# Autodesk Inventor assembly: 右後脚ユニット2
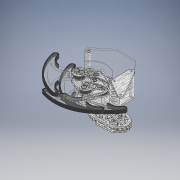
[picture p0: Inventor's stored thumbnail of the model, 180x180]
Saved by Autodesk Inventor 2020 (Build 240168000, 168)
## iProperties
Created: 2019-07-31
Part Number: 右後脚ユニット2
Document SubType Name: Assembly
Designer: 雪村
Mass: 201.521 g
Surface Area: 1076.65 cm^2
Volume: 97.0922 cm^3
Density: 2.07557 g/cm^3
Author: 雪村
## Documents named in this file (12)
- C:\Users\white\Documents\SRDC\SRDC\Inventor_2017\2018年機体\2020年4年機体\右後脚ユニット2.iam
- C:\Users\white\Documents\SRDC\SRDC\Inventor_2017\2018年機体\2020年4年機体\脚内フレーム1.ipt
- C:\Users\white\Documents\SRDC\SRDC\Inventor_2017\2018年機体\2020年4年機体\脚クランク1.iam
- C:\Users\white\Documents\SRDC\SRDC\Inventor_2017\2018年機体\パーツ\オイレスフランジ付き12142006.ipt
- C:\Users\white\Documents\SRDC\SRDC\Inventor_2017\2018年機体\2020年4年機体\脚最終段カム1.ipt
- C:\Users\white\Documents\SRDC\SRDC\Inventor_2017\2018年機体\2020年4年機体\歯車m2.z14.ipt
- C:\Users\white\Documents\SRDC\SRDC\Inventor_2017\2018年機体\パーツ\スペーサーm3,35.ipt
- C:\Users\white\Documents\SRDC\SRDC\Inventor_2017\2018年機体\2020年4年機体\ヘッケン＋揺動節1_MIR.iam
- C:\Users\white\Documents\SRDC\SRDC\Inventor_2017\2018年機体\2020年4年機体\脚外フレーム1.ipt
- C:\Users\white\Documents\SRDC\SRDC\Inventor_2017\2018年機体\2020年4年機体\後脚ギアトレイン1_MIR1.iam
- C:\Users\white\Documents\SRDC\SRDC\Inventor_2017\2018年機体\パーツ\オイレスフランジ付き14162202.5.ipt
- C:\Users\white\Documents\SRDC\SRDC\Inventor_2017\2018年機体\2020年4年機体\後脚ユニット締結パーツ2_MIR.ipt
## Components (16 placed, 11 different names)
1. 脚内フレーム1:1 — 挿入:9, 挿入:10, 挿入:11, 挿入:15, 挿入:18
2. 脚クランク1:1 [sub-assembly]
3. オイレスフランジ付き12142006:1 — 挿入:9
4. 脚最終段カム1:1
5. 歯車m2.z14:1
6. スペーサーm3,35:1 — 挿入:10, 挿入:13
7. スペーサーm3,35:2 — 挿入:11, 挿入:12
8. ヘッケン＋揺動節1_MIR:1 [sub-assembly]
9. ヘッケン＋揺動節1_MIR:2 [sub-assembly]
10. ヘッケン＋揺動節1_MIR:3 [sub-assembly]
11. ヘッケン＋揺動節1_MIR:4 [sub-assembly]
12. 脚外フレーム1:1 — 挿入:12, 挿入:13, 挿入:16, 挿入:17
13. 後脚ギアトレイン1_MIR1:1 [sub-assembly] — 挿入:14, メイト:6
14. オイレスフランジ付き14162202.5:1 — 挿入:14, 挿入:15
15. 後脚ユニット締結パーツ2_MIR:1 — 挿入:16, 挿入:17, メイト:6
16. スペーサーm3,35:3 — 挿入:18
## Relationships (24: Insert 18, Mate 6)
- [Insert]: 脚クランク1:1 ↔ 脚最終段カム1:1
- [Insert]: 脚クランク1:1 ↔ 脚最終段カム1:1
- [Insert]: オイレスフランジ付き12142006:1 ↔ 脚最終段カム1:1
- [Insert]: 脚最終段カム1:1 ↔ 歯車m2.z14:1
- [Mate]: 脚最終段カム1:1 ↔ 歯車m2.z14:1
- [Insert]: 脚クランク1:1 ↔ ヘッケン＋揺動節1_MIR:1
- [Insert]: 脚クランク1:1 ↔ ヘッケン＋揺動節1_MIR:2
- [Insert]: 脚クランク1:1 ↔ ヘッケン＋揺動節1_MIR:4
- [Insert]: 脚クランク1:1 ↔ ヘッケン＋揺動節1_MIR:3
- [Mate]: スペーサーm3,35:1 ↔ ヘッケン＋揺動節1_MIR:3
- [Mate]: スペーサーm3,35:1 ↔ ヘッケン＋揺動節1_MIR:4
- [Mate]: スペーサーm3,35:1 ↔ ヘッケン＋揺動節1_MIR:1
- [Mate]: スペーサーm3,35:1 ↔ ヘッケン＋揺動節1_MIR:2
- 挿入:9 [Insert]: 脚内フレーム1:1 ↔ オイレスフランジ付き12142006:1
- 挿入:10 [Insert]: 脚内フレーム1:1 ↔ スペーサーm3,35:1
- 挿入:11 [Insert]: 脚内フレーム1:1 ↔ スペーサーm3,35:2
- 挿入:12 [Insert]: スペーサーm3,35:2 ↔ 脚外フレーム1:1
- 挿入:13 [Insert]: スペーサーm3,35:1 ↔ 脚外フレーム1:1
- 挿入:14 [Insert]: 後脚ギアトレイン1_MIR1:1 ↔ オイレスフランジ付き14162202.5:1
- 挿入:15 [Insert]: 脚内フレーム1:1 ↔ オイレスフランジ付き14162202.5:1
- 挿入:16 [Insert]: 脚外フレーム1:1 ↔ 後脚ユニット締結パーツ2_MIR:1
- 挿入:17 [Insert]: 脚外フレーム1:1 ↔ 後脚ユニット締結パーツ2_MIR:1
- メイト:6 [Mate]: 後脚ギアトレイン1_MIR1:1 ↔ 後脚ユニット締結パーツ2_MIR:1
- 挿入:18 [Insert]: 脚内フレーム1:1 ↔ スペーサーm3,35:3
## Named parameters: d11_d12 = 0 mm
